# Autodesk Inventor assembly: R-SO v11
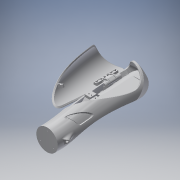
[picture p0: Inventor's stored thumbnail of the model, 180x180]
Saved by Autodesk Inventor 2018.2 (Build 222227000, 227)
## iProperties
Created: 2017-09-22
Part Number: R-SO v11
Material: 一般
Document SubType Name: Assembly
Designer: sktom
Author: sktom
## Documents named in this file (11)
- D:\CloudStrage\OneDrive\CADMech\HbSizeMMech\UnitSocket\Unit_MR-SO.iam
- D:\CloudStrage\OneDrive\CADMech\HbSizeMMech\UnitSocket\MR-SO-02.ipt
- D:\CloudStrage\OneDrive\CADMech\HbSizeMMech\UnitSocket\MR-SO-01.ipt
- D:\CloudStrage\OneDrive\CADMech\HbSizeMMech\UnitSocket\MR-SO-05.ipt
- D:\CloudStrage\OneDrive\CADMech\HbSizeMMech\UnitSocket\MR-SO-06.ipt
- D:\CloudStrage\OneDrive\CADMech\HbSizeMMech\UnitSocket\MR-SO-07.ipt
- D:\CloudStrage\OneDrive\CADMech\HbSizeMMech\UnitSocket\MR-SO-08.ipt
- D:\CloudStrage\OneDrive\CADMech\HbSizeMMech\UnitSocket\MR-SO-09.ipt
- D:\CloudStrage\OneDrive\CADMech\HbSizeMMech\UnitSocket\MR-SO-10.ipt
- D:\CloudStrage\OneDrive\CADMech\HbSizeMMech\UnitSocket\Parts_Screw_M2_L8.ipt
- D:\CloudStrage\OneDrive\CADMech\HbSizeMMech\UnitSocket\Parts_FlatScrew_M2_L6.ipt
## Components (21 placed, 10 different names)
1. MR-SO-01:1 — リジッド:2, 挿入:7, 挿入:11, 挿入:12
2. MR-SO-02:1 — リジッド:2, メイト:1, メイト:2, 挿入:9, 挿入:10, 挿入:13, 挿入:14
3. MR-SO-05:1 — メイト:1, メイト:2, メイト:3, メイト:4, メイト:5
4. MR-SO-06:1 — メイト:3, メイト:4, メイト:5, 挿入:8
5. MR-SO-07:1 — 挿入:1, 挿入:2, 挿入:3, 挿入:4, 挿入:5, 挿入:6, 挿入:7
6. MR-SO-08:1 — 挿入:5, 挿入:6, 挿入:19, 挿入:20
7. MR-SO-09:1 — 挿入:1, 挿入:2, 挿入:15, 挿入:16
8. MR-SO-10:1 — 挿入:3, 挿入:4, 挿入:17, 挿入:18
9. Parts_FlatScrew_M2_L6:1 — 挿入:15
10. Parts_FlatScrew_M2_L6:2 — 挿入:16
11. Parts_FlatScrew_M2_L6:3 — 挿入:17
12. Parts_FlatScrew_M2_L6:4 — 挿入:18
13. Parts_FlatScrew_M2_L6:5 — 挿入:19
14. Parts_FlatScrew_M2_L6:6 — 挿入:20
15. Parts_Screw_M2_L8:1 — 挿入:8
16. Parts_Screw_M2_L8:2 — 挿入:11
17. Parts_Screw_M2_L8:3 — 挿入:9
18. Parts_Screw_M2_L8:4 — 挿入:14
19. Parts_Screw_M2_L8:5 — 挿入:13
20. Parts_Screw_M2_L8:6 — 挿入:10
21. Parts_Screw_M2_L8:7 — 挿入:12
## Relationships (26: Insert 20, Mate 5, WeldJoint 1)
- リジッド:2 [WeldJoint] (-0.14 mm): MR-SO-01:1 ↔ MR-SO-02:1
- 挿入:1 [Insert]: MR-SO-07:1 ↔ MR-SO-09:1
- 挿入:2 [Insert]: MR-SO-07:1 ↔ MR-SO-09:1
- 挿入:3 [Insert]: MR-SO-07:1 ↔ MR-SO-10:1
- 挿入:4 [Insert]: MR-SO-07:1 ↔ MR-SO-10:1
- 挿入:5 [Insert]: MR-SO-07:1 ↔ MR-SO-08:1
- 挿入:6 [Insert]: MR-SO-07:1 ↔ MR-SO-08:1
- 挿入:7 [Insert] (0.2 mm): MR-SO-01:1 ↔ MR-SO-07:1
- メイト:1 [Mate] (0.1 mm): MR-SO-02:1 ↔ MR-SO-05:1
- メイト:2 [Mate] (0.1 mm): MR-SO-02:1 ↔ MR-SO-05:1
- メイト:3 [Mate]: MR-SO-05:1 ↔ MR-SO-06:1
- メイト:4 [Mate]: MR-SO-05:1 ↔ MR-SO-06:1
- メイト:5 [Mate]: MR-SO-05:1 ↔ MR-SO-06:1
- 挿入:8 [Insert]: MR-SO-06:1 ↔ Parts_Screw_M2_L8:1
- 挿入:9 [Insert]: MR-SO-02:1 ↔ Parts_Screw_M2_L8:3
- 挿入:10 [Insert]: MR-SO-02:1 ↔ Parts_Screw_M2_L8:6
- 挿入:11 [Insert]: MR-SO-01:1 ↔ Parts_Screw_M2_L8:2
- 挿入:12 [Insert]: MR-SO-01:1 ↔ Parts_Screw_M2_L8:7
- 挿入:13 [Insert]: MR-SO-02:1 ↔ Parts_Screw_M2_L8:5
- 挿入:14 [Insert]: MR-SO-02:1 ↔ Parts_Screw_M2_L8:4
- 挿入:15 [Insert]: MR-SO-09:1 ↔ Parts_FlatScrew_M2_L6:1
- 挿入:16 [Insert]: MR-SO-09:1 ↔ Parts_FlatScrew_M2_L6:2
- 挿入:17 [Insert]: MR-SO-10:1 ↔ Parts_FlatScrew_M2_L6:3
- 挿入:18 [Insert]: MR-SO-10:1 ↔ Parts_FlatScrew_M2_L6:4
- 挿入:19 [Insert]: MR-SO-08:1 ↔ Parts_FlatScrew_M2_L6:5
- 挿入:20 [Insert]: MR-SO-08:1 ↔ Parts_FlatScrew_M2_L6:6
